# Autodesk Inventor assembly: Walls
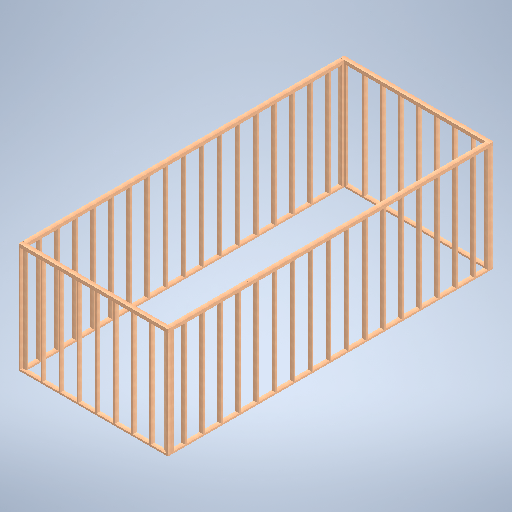
[picture p0: Inventor's stored thumbnail of the model, 512x512]
Saved by Autodesk Inventor 2025 (Build 290162010, 162A)
## iProperties
Created: 2024-09-15
Part Number: Walls
Document SubType Name: Assembly
Designer: Tom
Author: Tom
## Documents named in this file (7)
- C:\Users\Tom\Documents\Inventor\Mobility\Additional_Building\Walls.iam
- C:\Users\Tom\Documents\Inventor\Mobility\Additional_Building\Plate_With_Length_144_Inches.ipt
- C:\Users\Tom\Documents\Inventor\Mobility\Additional_Building\Plate_With_Length_125_Inches.ipt
- C:\Users\Tom\Documents\Inventor\Mobility\Additional_Building\California_Corner.iam
- C:\Users\Tom\Documents\Inventor\Mobility\Additional_Building\Stud_With_Height_93_Inches.ipt
- C:\Users\Tom\Documents\Inventor\Mobility\Additional_Building\Plate_With_Length_132_Inches.ipt
- C:\Users\Tom\Documents\Inventor\Mobility\Additional_Building\Plate_With_Length_68.5_Inches.ipt
## Components (72 placed, 6 different names)
1. California_Corner:1 [sub-assembly] — Mate:2, Flush:3, Flush:4
2. California_Corner:2 [sub-assembly] — Mate:13, Flush:13, Flush:14, Flush:19, Flush:20, Flush:21
3. California_Corner:3 [sub-assembly] — Mate:14, Flush:15, Flush:16
4. California_Corner:4 [sub-assembly] — Mate:15, Flush:17, Flush:18
5. Plate_With_Length_132_Inches:1 — Mate:8, Flush:9, Flush:10, Mate:10
6. Plate_With_Length_132_Inches:2
7. Plate_With_Length_144_Inches:9 — Mate:11, Mate:12, Flush:12
8. Plate_With_Length_144_Inches:10
9. Plate_With_Length_144_Inches:1 — Flush:5, Mate:15, Flush:17, Flush:18
10. Plate_With_Length_144_Inches:2 — Mate:14, Flush:15, Flush:16
11. Plate_With_Length_144_Inches:3 — Mate:1, Flush:1, Flush:2, Mate:4, Flush:6, Mate:13, Flush:13, Flush:14
12. Plate_With_Length_144_Inches:4 — Mate:2, Flush:3, Flush:4
13. Plate_With_Length_125_Inches:1 — Mate:1, Flush:1, Flush:2, Mate:3, Mate:7
14. Plate_With_Length_125_Inches:2
15. Plate_With_Length_144_Inches:5 — Flush:9
16. Plate_With_Length_144_Inches:6
17. Plate_With_Length_144_Inches:7 — Mate:9, Flush:11
18. Plate_With_Length_144_Inches:8 — Mate:11, Flush:12
19. Plate_With_Length_125_Inches:3 — Flush:7, Mate:8, Flush:10
20. Plate_With_Length_125_Inches:4
21. Stud_With_Height_93_Inches:1 — Mate:4, Flush:6, Flush:19
22. Stud_With_Height_93_Inches:2
23. Stud_With_Height_93_Inches:3
24. Stud_With_Height_93_Inches:4
25. Stud_With_Height_93_Inches:5
26. Stud_With_Height_93_Inches:6
27. Stud_With_Height_93_Inches:7
28. Stud_With_Height_93_Inches:8
29. Stud_With_Height_93_Inches:9
30. Stud_With_Height_93_Inches:10
31. Stud_With_Height_93_Inches:11
32. Stud_With_Height_93_Inches:33
33. Stud_With_Height_93_Inches:34
34. Stud_With_Height_93_Inches:35
35. Stud_With_Height_93_Inches:36
36. Stud_With_Height_93_Inches:37
37. Stud_With_Height_93_Inches:38
38. Stud_With_Height_93_Inches:12
39. Stud_With_Height_93_Inches:13
40. Stud_With_Height_93_Inches:14
41. Stud_With_Height_93_Inches:15
42. Stud_With_Height_93_Inches:16
43. Stud_With_Height_93_Inches:17
44. Stud_With_Height_93_Inches:18
45. Stud_With_Height_93_Inches:19
46. Stud_With_Height_93_Inches:20
47. Stud_With_Height_93_Inches:21
48. Stud_With_Height_93_Inches:22
49. Stud_With_Height_93_Inches:39
50. Stud_With_Height_93_Inches:40
51. Stud_With_Height_93_Inches:41
52. Stud_With_Height_93_Inches:42
53. Stud_With_Height_93_Inches:43
54. Stud_With_Height_93_Inches:44
55. Stud_With_Height_93_Inches:23 — Flush:7, Mate:7, Flush:20
56. Stud_With_Height_93_Inches:24
57. Stud_With_Height_93_Inches:25
58. Stud_With_Height_93_Inches:26
59. Stud_With_Height_93_Inches:27
60. Stud_With_Height_93_Inches:45
61. Stud_With_Height_93_Inches:46
62. Stud_With_Height_93_Inches:28
63. Stud_With_Height_93_Inches:29
64. Stud_With_Height_93_Inches:30
65. Stud_With_Height_93_Inches:31
66. Stud_With_Height_93_Inches:32
67. Stud_With_Height_93_Inches:47
68. Stud_With_Height_93_Inches:48
69. Plate_With_Length_68.5_Inches:1 — Mate:9, Mate:10, Flush:11
70. Plate_With_Length_68.5_Inches:2 — Mate:12
71. Plate_With_Length_68.5_Inches:3
72. Plate_With_Length_68.5_Inches:4
## Component patterns: (2 elements), (2 elements), (2 elements), (2 elements, first: Plate_With_Length_132_Inches:1), (2 elements, first: Plate_With_Length_144_Inches:9), (4 elements, first: Plate_With_Length_144_Inches:1), (2 elements, first: Plate_With_Length_125_Inches:1), Component Pattern 1:2 (4 elements), Component Pattern 2:2 (2 elements), (17 elements, first: Stud_With_Height_93_Inches:1), Component Pattern 4:2 (17 elements), (7 elements, first: Stud_With_Height_93_Inches:23), Component Pattern 6:2 (7 elements), (2 elements, first: Plate_With_Length_68.5_Inches:1), Component Pattern 10:2 (2 elements)
## Relationships (33: Flush 20, Mate 13)
- Mate:1: Plate_With_Length_144_Inches:3 ↔ Plate_With_Length_125_Inches:1
- Flush:1: Plate_With_Length_144_Inches:3 ↔ Plate_With_Length_125_Inches:1
- Flush:2: Plate_With_Length_144_Inches:3 ↔ Plate_With_Length_125_Inches:1
- Mate:2: California_Corner:1 ↔ Plate_With_Length_144_Inches:4
- Flush:3: California_Corner:1 ↔ Plate_With_Length_144_Inches:4
- Flush:4: California_Corner:1 ↔ Plate_With_Length_144_Inches:4
- Flush:5: Plate_With_Length_144_Inches:1
- Mate:3 (1536.7 mm): Plate_With_Length_125_Inches:1
- Mate:4: Plate_With_Length_144_Inches:3 ↔ Stud_With_Height_93_Inches:1
- Flush:6: Plate_With_Length_144_Inches:3 ↔ Stud_With_Height_93_Inches:1
- Flush:7: Plate_With_Length_125_Inches:3 ↔ Stud_With_Height_93_Inches:23
- Mate:7: Plate_With_Length_125_Inches:1 ↔ Stud_With_Height_93_Inches:23
- Mate:8: Plate_With_Length_132_Inches:1 ↔ Plate_With_Length_125_Inches:3
- Flush:9: Plate_With_Length_132_Inches:1 ↔ Plate_With_Length_144_Inches:5
- Flush:10: Plate_With_Length_132_Inches:1 ↔ Plate_With_Length_125_Inches:3
- Mate:9: Plate_With_Length_144_Inches:7 ↔ Plate_With_Length_68.5_Inches:1
- Mate:10: Plate_With_Length_132_Inches:1 ↔ Plate_With_Length_68.5_Inches:1
- Flush:11: Plate_With_Length_144_Inches:7 ↔ Plate_With_Length_68.5_Inches:1
- Mate:11: Plate_With_Length_144_Inches:9 ↔ Plate_With_Length_144_Inches:8
- Mate:12: Plate_With_Length_144_Inches:9 ↔ Plate_With_Length_68.5_Inches:2
- Flush:12: Plate_With_Length_144_Inches:9 ↔ Plate_With_Length_144_Inches:8
- Mate:13: California_Corner:2 ↔ Plate_With_Length_144_Inches:3
- Flush:13: California_Corner:2 ↔ Plate_With_Length_144_Inches:3
- Flush:14: California_Corner:2 ↔ Plate_With_Length_144_Inches:3
- Mate:14: California_Corner:3 ↔ Plate_With_Length_144_Inches:2
- Flush:15: California_Corner:3 ↔ Plate_With_Length_144_Inches:2
- Flush:16: California_Corner:3 ↔ Plate_With_Length_144_Inches:2
- Mate:15: California_Corner:4 ↔ Plate_With_Length_144_Inches:1
- Flush:17: California_Corner:4 ↔ Plate_With_Length_144_Inches:1
- Flush:18: California_Corner:4 ↔ Plate_With_Length_144_Inches:1
- Flush:19 (387.35 mm): California_Corner:2 ↔ Stud_With_Height_93_Inches:1
- Flush:20 (492.125 mm): California_Corner:2 ↔ Stud_With_Height_93_Inches:23
- Flush:21 (15.875 mm): California_Corner:2
